# Autodesk Inventor assembly: Skirt Fan-Assembly
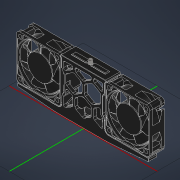
[picture p0: Inventor's stored thumbnail of the model, 180x180]
Saved by Autodesk Inventor 2022.2 (Build 262287010, 287A)
## iProperties
Created: 2022-03-13
Part Number: Skirt Fan-Assembly
Document SubType Name: Assembly
Designer: sleib
Author: sleib
## Documents named in this file (6)
- C:\Users\sleib\Projekte\Voron-2\CAD\Inventor\Skirt Fan-Assembly.iam
- C:\Users\sleib\Projekte\Voron-2\CAD\Inventor\Skirt Fan-Support.ipt
- C:\Users\sleib\Projekte\Voron-2\CAD\Inventor\M5x10 BHCS.ipt
- C:\Users\sleib\Projekte\Voron-2\CAD\Inventor\Fan 6020.iam
- C:\Users\sleib\Projekte\Voron-2\CAD\Inventor\Tape VHB Fan.ipt
- C:\Users\sleib\Projekte\Voron-2\CAD\Inventor\M3 Threaded Insert.ipt
## Components (11 placed, 5 different names)
1. Skirt Fan-Support:1 — Passend:1, Passend:2, Passend:8, Passend:9, Fluchtend:4, Passend:13, Passend:14, Fluchtend:8, Fluchtend:9, Passend:15, Passend:16, Passend:17, Passend:18, Fluchtend:10
2. M5x10 BHCS:1 — Passend:1, Passend:2
3. Fan 6020:1 [sub-assembly] — Passend:5, Fluchtend:1, Tangential:1, Passend:6, Fluchtend:2, Tangential:2, Passend:7, Fluchtend:3, Tangential:3, Fluchtend:4
4. Fan 6020:2 [sub-assembly] — Passend:10, Passend:11, Passend:12, Fluchtend:5, Fluchtend:6, Fluchtend:7, Tangential:4, Tangential:5, Tangential:6, Fluchtend:8
5. Tape VHB Fan:1 — Passend:5, Fluchtend:1, Tangential:1
6. Tape VHB Fan:2 — Passend:6, Fluchtend:2, Tangential:2, Passend:8
7. Tape VHB Fan:3 — Passend:7, Fluchtend:3, Tangential:3, Passend:9
8. Tape VHB Fan:4 — Passend:10, Fluchtend:7, Tangential:4
9. Tape VHB Fan:5 — Passend:11, Fluchtend:6, Tangential:5, Passend:13
10. Tape VHB Fan:6 — Passend:12, Fluchtend:5, Tangential:6, Passend:14
11. M3 Threaded Insert:1 — Passend:18, Fluchtend:10
## Relationships (32: Mate 16, Flush 10, Tangent 6)
- Passend:1 [Mate]: Skirt Fan-Support:1 ↔ M5x10 BHCS:1
- Passend:2 [Mate]: Skirt Fan-Support:1 ↔ M5x10 BHCS:1
- Passend:5 [Mate]: Fan 6020:1 ↔ Tape VHB Fan:1
- Fluchtend:1 [Flush]: Fan 6020:1 ↔ Tape VHB Fan:1
- Tangential:1: Fan 6020:1 ↔ Tape VHB Fan:1
- Passend:6 [Mate]: Fan 6020:1 ↔ Tape VHB Fan:2
- Fluchtend:2 [Flush]: Fan 6020:1 ↔ Tape VHB Fan:2
- Tangential:2: Fan 6020:1 ↔ Tape VHB Fan:2
- Passend:7 [Mate]: Fan 6020:1 ↔ Tape VHB Fan:3
- Fluchtend:3 [Flush]: Fan 6020:1 ↔ Tape VHB Fan:3
- Tangential:3: Fan 6020:1 ↔ Tape VHB Fan:3
- Passend:8 [Mate]: Skirt Fan-Support:1 ↔ Tape VHB Fan:2
- Passend:9 [Mate]: Skirt Fan-Support:1 ↔ Tape VHB Fan:3
- Fluchtend:4 [Flush]: Skirt Fan-Support:1 ↔ Fan 6020:1
- Passend:10 [Mate]: Fan 6020:2 ↔ Tape VHB Fan:4
- Passend:11 [Mate]: Fan 6020:2 ↔ Tape VHB Fan:5
- Passend:12 [Mate]: Fan 6020:2 ↔ Tape VHB Fan:6
- Fluchtend:5 [Flush]: Fan 6020:2 ↔ Tape VHB Fan:6
- Fluchtend:6 [Flush]: Fan 6020:2 ↔ Tape VHB Fan:5
- Fluchtend:7 [Flush]: Fan 6020:2 ↔ Tape VHB Fan:4
- Tangential:4: Fan 6020:2 ↔ Tape VHB Fan:4
- Tangential:5: Fan 6020:2 ↔ Tape VHB Fan:5
- Tangential:6: Fan 6020:2 ↔ Tape VHB Fan:6
- Passend:13 [Mate]: Skirt Fan-Support:1 ↔ Tape VHB Fan:5
- Passend:14 [Mate]: Skirt Fan-Support:1 ↔ Tape VHB Fan:6
- Fluchtend:8 [Flush]: Skirt Fan-Support:1 ↔ Fan 6020:2
- Fluchtend:9 [Flush]: Skirt Fan-Support:1
- Passend:15 [Mate]: Skirt Fan-Support:1
- Passend:16 [Mate]: Skirt Fan-Support:1
- Passend:17 [Mate]: Skirt Fan-Support:1
- Passend:18 [Mate]: Skirt Fan-Support:1 ↔ M3 Threaded Insert:1
- Fluchtend:10 [Flush]: Skirt Fan-Support:1 ↔ M3 Threaded Insert:1
